# Autodesk Inventor assembly: trzymak
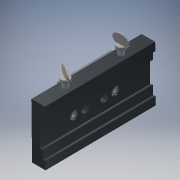
[picture p0: Inventor's stored thumbnail of the model, 180x180]
Saved by Autodesk Inventor 2019 (Build 230136000, 136)
## iProperties
Created: 2020-08-30
Part Number: trzymak
Document SubType Name: Assembly
Designer: estee
Author: estee
## Documents named in this file (7)
- C:\Users\estee\OneDrive\Pulpit\estere\1\MUM\wogoleNajnowszyGit\Mechanika\Moduł obrotu RET Estera\projejt\projejt\Zlozenie\trzymak.iam
- C:\Users\estee\OneDrive\Pulpit\estere\1\MUM\wogoleNajnowszyGit\Mechanika\Moduł obrotu RET Estera\projejt\projejt\Zlozenie\plytkaadaptacyjna.ipt
- C:\Users\estee\OneDrive\Pulpit\estere\1\MUM\wogoleNajnowszyGit\Mechanika\Moduł obrotu RET Estera\projejt\projejt\Zlozenie\uchwytDoSzyny.iam
- C:\Users\estee\OneDrive\Pulpit\estere\1\MUM\wogoleNajnowszyGit\Mechanika\Moduł obrotu RET Estera\projejt\projejt\Zlozenie\kolnierz.ipt
- C:\Users\estee\OneDrive\Dokumenty\Inventor\Content Center Files\R2019\en-US\ISO 4762(2)\ISO 4762 - M8 x 20ISO.ipt
- C:\Users\estee\OneDrive\Dokumenty\Inventor\Content Center Files\R2019\en-US\ISO 4032(2)\ISO 4032 - M8 - ISO.ipt
- C:\Users\estee\OneDrive\Dokumenty\Inventor\Content Center Files\R2019\en-US\ISO 7046-1 Z(1)\ISO 7046-1 - M3 x 8 - 4.8 - Z - ISO.ipt
## Components (11 placed, 6 different names)
1. plytkaadaptacyjna:1 — Mate:1, Mate:2, Mate:3, Mate:12, Mate:13, Mate:14, Mate:19, Mate:20, Mate:23, Mate:24, Mate:25, Mate:26, Flush:1, Flush:2, Flush:3, Flush:4
2. uchwytDoSzyny:1 [sub-assembly] — Mate:12, Mate:13, Mate:14, Mate:15, Mate:16, Mate:17, Mate:18
3. kolnierz:2 — Mate:1, Mate:2, Mate:3
4. ISO 4762 M8 x 20:1 — Mate:17, Mate:18, Mate:22
5. ISO 4762 M8 x 20:2 — Mate:15, Mate:16, Mate:21
6. ISO 4032 M8:1 — Mate:19, Mate:22
7. ISO 4032 M8:2 — Mate:20, Mate:21
8. ISO 7046-1 Z M3 x 8 - 4.8 - Z:2 — Mate:23, Flush:1
9. ISO 7046-1 Z M3 x 8 - 4.8 - Z:3 — Mate:25, Flush:4
10. ISO 7046-1 Z M3 x 8 - 4.8 - Z:4 — Mate:26, Flush:2
11. ISO 7046-1 Z M3 x 8 - 4.8 - Z:5 — Mate:24, Flush:3
## Relationships (22: Mate 18, Flush 4)
- Mate:1: plytkaadaptacyjna:1 ↔ kolnierz:2
- Mate:2: plytkaadaptacyjna:1 ↔ kolnierz:2
- Mate:3: plytkaadaptacyjna:1 ↔ kolnierz:2
- Mate:12: plytkaadaptacyjna:1 ↔ uchwytDoSzyny:1
- Mate:13: plytkaadaptacyjna:1 ↔ uchwytDoSzyny:1
- Mate:14: plytkaadaptacyjna:1 ↔ uchwytDoSzyny:1
- Mate:15: uchwytDoSzyny:1 ↔ ISO 4762 M8 x 20:2
- Mate:16: uchwytDoSzyny:1 ↔ ISO 4762 M8 x 20:2
- Mate:17: uchwytDoSzyny:1 ↔ ISO 4762 M8 x 20:1
- Mate:18: uchwytDoSzyny:1 ↔ ISO 4762 M8 x 20:1
- Mate:19: plytkaadaptacyjna:1 ↔ ISO 4032 M8:1
- Mate:20: plytkaadaptacyjna:1 ↔ ISO 4032 M8:2
- Mate:21: ISO 4762 M8 x 20:2 ↔ ISO 4032 M8:2
- Mate:22: ISO 4762 M8 x 20:1 ↔ ISO 4032 M8:1
- Mate:23: plytkaadaptacyjna:1 ↔ ISO 7046-1 Z M3 x 8 - 4.8 - Z:2
- Mate:24: plytkaadaptacyjna:1 ↔ ISO 7046-1 Z M3 x 8 - 4.8 - Z:5
- Mate:25: plytkaadaptacyjna:1 ↔ ISO 7046-1 Z M3 x 8 - 4.8 - Z:3
- Mate:26: plytkaadaptacyjna:1 ↔ ISO 7046-1 Z M3 x 8 - 4.8 - Z:4
- Flush:1: plytkaadaptacyjna:1 ↔ ISO 7046-1 Z M3 x 8 - 4.8 - Z:2
- Flush:2: plytkaadaptacyjna:1 ↔ ISO 7046-1 Z M3 x 8 - 4.8 - Z:4
- Flush:3: plytkaadaptacyjna:1 ↔ ISO 7046-1 Z M3 x 8 - 4.8 - Z:5
- Flush:4: plytkaadaptacyjna:1 ↔ ISO 7046-1 Z M3 x 8 - 4.8 - Z:3
